# Autodesk Inventor assembly: Assembly_LampeSolaire2_v2
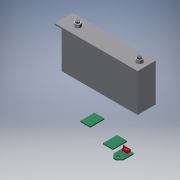
[picture p0: Inventor's stored thumbnail of the model, 180x180]
Saved by Autodesk Inventor 2019 (Build 230136000, 136)
## iProperties
Created: 2020-12-17
Part Number: Assembly_LampeSolaire2_v2
Document SubType Name: Assembly
Designer: nicolas
Author: nicolas
## Documents named in this file (11)
- C:\Workspace\3D\Cad\LampeSolaire2\Assembly_LampeSolaire2_v2.iam
- C:\Workspace\3D\Cad\LampeSolaire2\ChargerModule.iam
- C:\Workspace\3D\Cad\LampeSolaire2\LampeSolaire2.iam
- C:\Workspace\3D\Cad\LampeSolaire2\ledsAdapter_base.ipt
- C:\Workspace\3D\Cad\LampeSolaire2\LedAdapter.ipt
- C:\Workspace\3D\Cad\Screws\Hex_m5\M5x0.8xL.ipt
- C:\Workspace\3D\Cad\Nuts\Nut_Generic\Ec 6p ISO 4032-M5.ipt
- C:\Workspace\3D\Cad\Nuts\Nut_Generic.ipt
- C:\Workspace\3D\Cad\Casings\Casing_1.ipt
- C:\Workspace\3D\Cad\Screws\Hex_m5\M5x0.8xL\M5x0.8x60.ipt
- C:\Workspace\3D\Cad\Casings\Casing_2.ipt
## Components (17 placed, 8 different names)
1. ChargerModule:1 [sub-assembly] — Mate:17, Mate:18, Mate:19, Mate:20, Cylindrical:5
2. LampeSolaire2:1 [sub-assembly] — Mate:9, Mate:10, Cylindrical:4, Mate:14, Mate:15, Mate:16, Mate:20
3. ledsAdapter_base:1
4. LedAdapter:1
5. LedAdapter:2
6. M5x0.8x60:1 — Mate:1, Mate:2, Flush:1, Cylindrical:1, Cylindrical:2, Mate:9, Mate:12, Mate:18, Mate:21, Mate:23, Mate:25, Mate:28
7. M5x0.8x60:2 — Mate:3, Mate:4, Flush:1, Mate:10, Mate:13, Mate:17, Mate:22, Mate:24, Mate:27
8. Ec 6p ISO 4032-M5:1 — Mate:1, Cylindrical:1, Cylindrical:3, Mate:19, Flush:3
9. Ec 6p ISO 4032-M5:2 — Mate:2, Cylindrical:2, Cylindrical:3, Flush:2, Cylindrical:4
10. Ec 6p ISO 4032-M5:3 — Mate:3, Flush:2, Mate:16
11. Ec 6p ISO 4032-M5:4 — Mate:4, Flush:3
12. Ec 6p ISO 4032-M5:5 — Mate:12, Mate:14
13. Ec 6p ISO 4032-M5:6 — Mate:13, Mate:15
14. Casing_1:1 — Mate:21, Mate:22, Mate:23, Cylindrical:5, Mate:26
15. Casing_2:1 — Mate:24, Mate:25, Mate:26, Mate:29, Mate:30
16. Ec 6p ISO 4032-M5:7 — Mate:28, Mate:30
17. Ec 6p ISO 4032-M5:8 — Mate:27, Mate:29
## Relationships (33: Mate 25, CylindricalJoint 5, Flush 3)
- Mate:1: M5x0.8x60:1 ↔ Ec 6p ISO 4032-M5:1
- Mate:2: M5x0.8x60:1 ↔ Ec 6p ISO 4032-M5:2
- Mate:3: M5x0.8x60:2 ↔ Ec 6p ISO 4032-M5:3
- Mate:4: M5x0.8x60:2 ↔ Ec 6p ISO 4032-M5:4
- Flush:1: M5x0.8x60:1 ↔ M5x0.8x60:2
- Cylindrical:1: M5x0.8x60:1 ↔ Ec 6p ISO 4032-M5:1
- Cylindrical:2: M5x0.8x60:1 ↔ Ec 6p ISO 4032-M5:2
- Cylindrical:3: Ec 6p ISO 4032-M5:1 ↔ Ec 6p ISO 4032-M5:2
- Flush:2: Ec 6p ISO 4032-M5:2 ↔ Ec 6p ISO 4032-M5:3
- Mate:9: LampeSolaire2:1 ↔ M5x0.8x60:1
- Mate:10: LampeSolaire2:1 ↔ M5x0.8x60:2
- Cylindrical:4: LampeSolaire2:1 ↔ Ec 6p ISO 4032-M5:2
- Mate:12: M5x0.8x60:1 ↔ Ec 6p ISO 4032-M5:5
- Mate:13: M5x0.8x60:2 ↔ Ec 6p ISO 4032-M5:6
- Mate:14: LampeSolaire2:1 ↔ Ec 6p ISO 4032-M5:5
- Mate:15: LampeSolaire2:1 ↔ Ec 6p ISO 4032-M5:6
- Mate:16: LampeSolaire2:1 ↔ Ec 6p ISO 4032-M5:3
- Mate:17: ChargerModule:1 ↔ M5x0.8x60:2
- Mate:18: ChargerModule:1 ↔ M5x0.8x60:1
- Mate:19: ChargerModule:1 ↔ Ec 6p ISO 4032-M5:1
- Flush:3: Ec 6p ISO 4032-M5:1 ↔ Ec 6p ISO 4032-M5:4
- Mate:20: ChargerModule:1 ↔ LampeSolaire2:1
- Mate:21: M5x0.8x60:1 ↔ Casing_1:1
- Mate:22: M5x0.8x60:2 ↔ Casing_1:1
- Mate:23: M5x0.8x60:1 ↔ Casing_1:1
- Cylindrical:5: ChargerModule:1 ↔ Casing_1:1
- Mate:24: M5x0.8x60:2 ↔ Casing_2:1
- Mate:25: M5x0.8x60:1 ↔ Casing_2:1
- Mate:26: Casing_1:1 ↔ Casing_2:1
- Mate:27: M5x0.8x60:2 ↔ Ec 6p ISO 4032-M5:8
- Mate:28: M5x0.8x60:1 ↔ Ec 6p ISO 4032-M5:7
- Mate:29: Casing_2:1 ↔ Ec 6p ISO 4032-M5:8
- Mate:30: Casing_2:1 ↔ Ec 6p ISO 4032-M5:7
